# Autodesk Inventor assembly: Dead Axle Tensioner
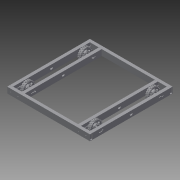
[picture p0: Inventor's stored thumbnail of the model, 180x180]
Saved by Autodesk Inventor 2015 SP1 (Build 190203100, 203)
## iProperties
Created: 2014-12-28
Part Number: Dead Axle Tensioner
Document SubType Name: Assembly
Designer: Jarod
Author: Jarod
## Documents named in this file (7)
- C:\Users\Jarod\Documents\Westview\Robotics\FRC\2015\CAD\Ideas\Dead Axle Tensioner\Dead Axle Tensioner.iam
- C:\Users\Jarod\Documents\Westview\Robotics\FRC\2015\CAD\Ideas\Dead Axle Tensioner\frame_long.ipt
- C:\Users\Jarod\Documents\Westview\Robotics\FRC\2015\CAD\Ideas\Dead Axle Tensioner\frame_wide.ipt
- C:\Users\Jarod\Documents\Westview\Robotics\FRC\2015\CAD\Ideas\Dead Axle Tensioner\dead_axle.ipt
- C:\Users\Jarod\Documents\Westview\Robotics\FRC\2015\CAD\Ideas\Dead Axle Tensioner\tension_block.ipt
- C:\Users\Jarod\Documents\Westview\Robotics\FRC\2015\CAD\Ideas\Dead Axle Tensioner\tension_bolt.ipt
- C:\Users\Jarod\Documents\Westview\Robotics\FRC\2015\CAD\Ideas\Dead Axle Tensioner\Imported Components\4 in HiGrip Wheel\4 in HiGrip Wheel.iam
## Components (26 placed, 6 different names)
1. frame_long:1 — Flush:1, Flush:5, Mate:1, Mate:5, Flush:6, Flush:8, Mate:7, Mate:8, Mate:9, Mate:10, Mate:11, Mate:49, Flush:9, Flush:10
2. frame_long:2 — Flush:2, Mate:2, Mate:7
3. frame_long:3 — Flush:3, Mate:3, Mate:6
4. frame_long:4 — Flush:4, Mate:4, Flush:7, Mate:6, Mate:12, Mate:13, Mate:14, Mate:15
5. frame_wide:1 — Flush:1, Flush:2, Flush:3, Flush:4, Mate:1, Mate:2, Mate:3, Mate:4, Flush:6, Flush:7, Mate:16, Mate:19, Mate:20, Mate:21, Mate:24, Mate:26, Mate:28, Mate:32, Mate:38, Mate:40, Mate:43
6. frame_wide:2 — Flush:5, Mate:5, Flush:8, Mate:17, Mate:18, Mate:22, Mate:23, Mate:25, Mate:27, Mate:36, Mate:37, Mate:45, Mate:46
7. dead_axle:1 — Mate:8, Mate:9, Mate:31, Mate:39, Mate:41, Mate:50
8. dead_axle:2 — Mate:10, Mate:11, Mate:30, Mate:48, Mate:51
9. dead_axle:3 — Mate:12, Mate:13, Mate:33, Mate:42, Mate:52
10. dead_axle:4 — Mate:14, Mate:15, Mate:35, Mate:47, Mate:53
11. tension_block:1 — Mate:16, Mate:21, Mate:24
12. tension_block:2 — Mate:17, Mate:22, Mate:25
13. tension_block:3 — Mate:19, Mate:20, Mate:26
14. tension_block:4 — Mate:18, Mate:23, Mate:27
15. tension_bolt:1 — Mate:28, Mate:31, Mate:38, Mate:39
16. tension_bolt:2 — Mate:30, Mate:36
17. tension_bolt:3 — Mate:32, Mate:33
18. tension_bolt:4 — Mate:35, Mate:37
19. tension_bolt:5 — Mate:40, Mate:41
20. tension_bolt:6 — Mate:46, Mate:48
21. tension_bolt:7 — Mate:42, Mate:43
22. tension_bolt:8 — Mate:45, Mate:47
23. 4 in HiGrip Wheel:1 [sub-assembly] — Mate:50
24. 4 in HiGrip Wheel:2 [sub-assembly] — Mate:51
25. 4 in HiGrip Wheel:3 [sub-assembly] — Mate:52
26. 4 in HiGrip Wheel:4 [sub-assembly] — Mate:53
## Relationships (60: Mate 50, Flush 10)
- Flush:1: frame_long:1 ↔ frame_wide:1
- Flush:2: frame_long:2 ↔ frame_wide:1
- Flush:3: frame_long:3 ↔ frame_wide:1
- Flush:4: frame_long:4 ↔ frame_wide:1
- Flush:5: frame_long:1 ↔ frame_wide:2
- Mate:1: frame_long:1 ↔ frame_wide:1
- Mate:2: frame_long:2 ↔ frame_wide:1
- Mate:3: frame_long:3 ↔ frame_wide:1
- Mate:4: frame_long:4 ↔ frame_wide:1
- Mate:5: frame_long:1 ↔ frame_wide:2
- Flush:6: frame_long:1 ↔ frame_wide:1
- Flush:7: frame_long:4 ↔ frame_wide:1
- Flush:8: frame_long:1 ↔ frame_wide:2
- Mate:6 (76.2 mm): frame_long:3 ↔ frame_long:4
- Mate:7 (76.2 mm): frame_long:1 ↔ frame_long:2
- Mate:8: frame_long:1 ↔ dead_axle:1
- Mate:9: frame_long:1 ↔ dead_axle:1
- Mate:10: frame_long:1 ↔ dead_axle:2
- Mate:11: frame_long:1 ↔ dead_axle:2
- Mate:12: frame_long:4 ↔ dead_axle:3
- Mate:13: frame_long:4 ↔ dead_axle:3
- Mate:14: frame_long:4 ↔ dead_axle:4
- Mate:15: frame_long:4 ↔ dead_axle:4
- Mate:16: frame_wide:1 ↔ tension_block:1
- Mate:17: frame_wide:2 ↔ tension_block:2
- Mate:18: frame_wide:2 ↔ tension_block:4
- Mate:19: frame_wide:1 ↔ tension_block:3
- Mate:20: frame_wide:1 ↔ tension_block:3
- Mate:21: frame_wide:1 ↔ tension_block:1
- Mate:22: frame_wide:2 ↔ tension_block:2
- Mate:23: frame_wide:2 ↔ tension_block:4
- Mate:24: frame_wide:1 ↔ tension_block:1
- Mate:25: frame_wide:2 ↔ tension_block:2
- Mate:26: frame_wide:1 ↔ tension_block:3
- Mate:27: frame_wide:2 ↔ tension_block:4
- Mate:28: frame_wide:1 ↔ tension_bolt:1
- Mate:30: dead_axle:2 ↔ tension_bolt:2
- Mate:31: dead_axle:1 ↔ tension_bolt:1
- Mate:32: frame_wide:1 ↔ tension_bolt:3
- Mate:33: dead_axle:3 ↔ tension_bolt:3
- Mate:35: dead_axle:4 ↔ tension_bolt:4
- Mate:36: frame_wide:2 ↔ tension_bolt:2
- Mate:37: frame_wide:2 ↔ tension_bolt:4
- Mate:38: frame_wide:1 ↔ tension_bolt:1
- Mate:39: dead_axle:1 ↔ tension_bolt:1
- Mate:40: frame_wide:1 ↔ tension_bolt:5
- Mate:41: dead_axle:1 ↔ tension_bolt:5
- Mate:42: dead_axle:3 ↔ tension_bolt:7
- Mate:43: frame_wide:1 ↔ tension_bolt:7
- Mate:45: frame_wide:2 ↔ tension_bolt:8
- Mate:46: frame_wide:2 ↔ tension_bolt:6
- Mate:47: dead_axle:4 ↔ tension_bolt:8
- Mate:48: dead_axle:2 ↔ tension_bolt:6
- Mate:49: frame_long:1
- Mate:50: dead_axle:1 ↔ 4 in HiGrip Wheel:1
- Mate:51: dead_axle:2 ↔ 4 in HiGrip Wheel:2
- Mate:52: dead_axle:3 ↔ 4 in HiGrip Wheel:3
- Mate:53: dead_axle:4 ↔ 4 in HiGrip Wheel:4
- Flush:9: frame_long:1
- Flush:10: frame_long:1
